# Autodesk Inventor assembly: RTrident
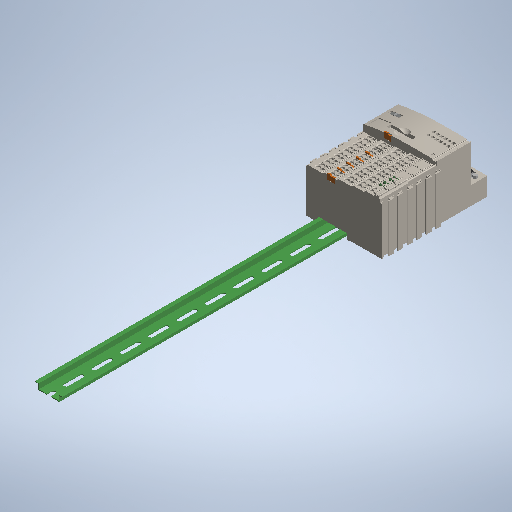
[picture p0: Inventor's stored thumbnail of the model, 512x512]
Saved by Autodesk Inventor 2025.4 (Build 294407000, 407)
## iProperties
Company: CADENAS
Created: 2026-05-16
Part Number: RTrident
Description: STEP AP242
Document SubType Name: Assembly
Designer: louis
Sending System: PARTsolutions
Preprocessor: ST-DEVELOPER v20
Title: RTrident
Author: License CC BY-ND 4.0
## Documents named in this file (6)
- C:\Users\louis\OneDrive\Desktop\R_Trident\02_CAD\01_Standard_Parts\Electrical_Automation\WAGO_Din.iam
- C:\Users\louis\OneDrive\Desktop\R_Trident\02_CAD\01_Standard_Parts\Electrical_Automation\WAGO_210-112500.ipt
- C:\Users\louis\OneDrive\Desktop\R_Trident\02_CAD\01_Standard_Parts\Electrical_Automation\750-8212.ipt
- C:\Users\louis\OneDrive\Desktop\R_Trident\02_CAD\01_Standard_Parts\Electrical_Automation\750-530.ipt
- C:\Users\louis\OneDrive\Desktop\R_Trident\02_CAD\01_Standard_Parts\Electrical_Automation\750-408.ipt
- C:\Users\louis\OneDrive\Desktop\R_Trident\02_CAD\01_Standard_Parts\Electrical_Automation\750-600.ipt
## Components (7 placed, 7 different names)
1. NAUO1 — Flush:1
2. NAUO2
3. NAUO3
4. NAUO4
5. NAUO5
6. NAUO6
7. NAUO7
## Relationships (1: Flush 1)
- Flush:1 (-250 mm): NAUO1
